# Autodesk Inventor assembly: Diffusion_dryer
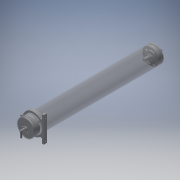
[picture p0: Inventor's stored thumbnail of the model, 180x180]
Saved by Autodesk Inventor 2016 (Build 200138000, 138)
## iProperties
Created: 2016-10-17
Part Number: Diffusion_dryer
Document SubType Name: Assembly
Designer: rawrdong
Author: rawrdong
## Documents named in this file (8)
- C:\Users\rawrdong\Box Sync\0_GradSchoolResearch\00_projects\0_AirParticleCounter\NEW_SHIT\NEBULIZER\Diffusion_dryer.iam
- C:\Users\rawrdong\Box Sync\0_GradSchoolResearch\00_projects\0_AirParticleCounter\NEW_SHIT\NEBULIZER\inner.ipt
- C:\Users\rawrdong\Box Sync\0_GradSchoolResearch\00_projects\0_AirParticleCounter\NEW_SHIT\NEBULIZER\cap.ipt
- C:\Users\rawrdong\Box Sync\0_GradSchoolResearch\00_projects\0_AirParticleCounter\NEW_SHIT\NEBULIZER\tube.ipt
- C:\Users\rawrdong\Box Sync\0_GradSchoolResearch\00_projects\0_AirParticleCounter\NEW_SHIT\NEBULIZER\mcmaster\5372K112_DURABLE NYLON EXTRA-GRIP BARBED TUBE FITTING.ipt
- C:\Users\rawrdong\Box Sync\0_GradSchoolResearch\00_projects\0_AirParticleCounter\NEW_SHIT\NEBULIZER\mcmaster\5372K312_DURABLE NYLON EXTRA-GRIP BARBED TUBE FITTING.ipt
- C:\Users\rawrdong\Box Sync\0_GradSchoolResearch\00_projects\0_AirParticleCounter\NEW_SHIT\NEBULIZER\mcmaster\5372K123_DURABLE NYLON EXTRA-GRIP BARBED TUBE FITTING.ipt
- C:\Users\rawrdong\Box Sync\0_GradSchoolResearch\00_projects\0_AirParticleCounter\NEW_SHIT\NEBULIZER\mount.ipt
## Components (10 placed, 7 different names)
1. inner:1 — Mate:7, Mate:10
2. cap:1 — Mate:1, Mate:2
3. tube:1 — Mate:3, Mate:4, Flush:1
4. 5372K112_DURABLE NYLON EXTRA-GRIP BARBED TUBE FITTING:1 — Mate:5, Mate:6
5. 5372K312_DURABLE NYLON EXTRA-GRIP BARBED TUBE FITTING:1 — Mate:1, Mate:2
6. inner:2 — Mate:3, Mate:8, Mate:9
7. cap:2 — Mate:4, Mate:5, Mate:6, Flush:1
8. 5372K123_DURABLE NYLON EXTRA-GRIP BARBED TUBE FITTING:1 — Mate:7, Mate:10
9. 5372K123_DURABLE NYLON EXTRA-GRIP BARBED TUBE FITTING:2 — Mate:8, Mate:9
10. mount:1
## Relationships (11: Mate 10, Flush 1)
- Mate:1: cap:1 ↔ 5372K312_DURABLE NYLON EXTRA-GRIP BARBED TUBE FITTING:1
- Mate:2: cap:1 ↔ 5372K312_DURABLE NYLON EXTRA-GRIP BARBED TUBE FITTING:1
- Mate:3: tube:1 ↔ inner:2
- Mate:4: tube:1 ↔ cap:2
- Mate:5: 5372K112_DURABLE NYLON EXTRA-GRIP BARBED TUBE FITTING:1 ↔ cap:2
- Mate:6: 5372K112_DURABLE NYLON EXTRA-GRIP BARBED TUBE FITTING:1 ↔ cap:2
- Flush:1: tube:1 ↔ cap:2
- Mate:7: inner:1 ↔ 5372K123_DURABLE NYLON EXTRA-GRIP BARBED TUBE FITTING:1
- Mate:8: inner:2 ↔ 5372K123_DURABLE NYLON EXTRA-GRIP BARBED TUBE FITTING:2
- Mate:9: inner:2 ↔ 5372K123_DURABLE NYLON EXTRA-GRIP BARBED TUBE FITTING:2
- Mate:10: inner:1 ↔ 5372K123_DURABLE NYLON EXTRA-GRIP BARBED TUBE FITTING:1
